# Autodesk Inventor assembly: my trunk assembly_MIR
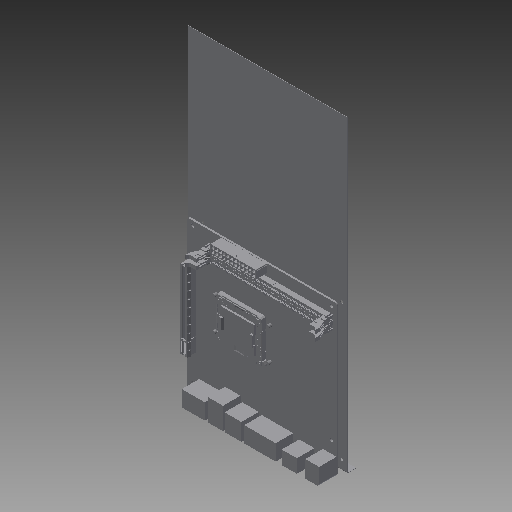
[picture p0: Inventor's stored thumbnail of the model, 512x512]
Saved by Autodesk Inventor 2018 (Build 220112000, 112)
## iProperties
Created: 2018-06-19
Part Number: my trunk assembly_MIR
Document SubType Name: Assembly
Designer: John Viljoen
Author: John Viljoen
## Documents named in this file (3)
- C:\Users\John Viljoen\Documents\Inventor\computer project\my trunk assembly_MIR.iam
- C:\Users\John Viljoen\Documents\Inventor\computer project\my trunk_MIR.ipt
- C:\Users\John Viljoen\Documents\Inventor\computer project\Mini-ITX Mobo_MIR.ipt
## Components (2 placed, 2 different names)
1. my trunk_MIR:1 — Flush:2, Flush:1, Mate:1
2. Mini-ITX Mobo_MIR:1 — Flush:2, Flush:1, Mate:1
## Relationships (3: Flush 2, Mate 1)
- Flush:2: my trunk_MIR:1 ↔ Mini-ITX Mobo_MIR:1
- Flush:1 (3 mm): my trunk_MIR:1 ↔ Mini-ITX Mobo_MIR:1
- Mate:1 (10 mm): my trunk_MIR:1 ↔ Mini-ITX Mobo_MIR:1
